# Autodesk Inventor assembly: LIA0002-LID ASSY
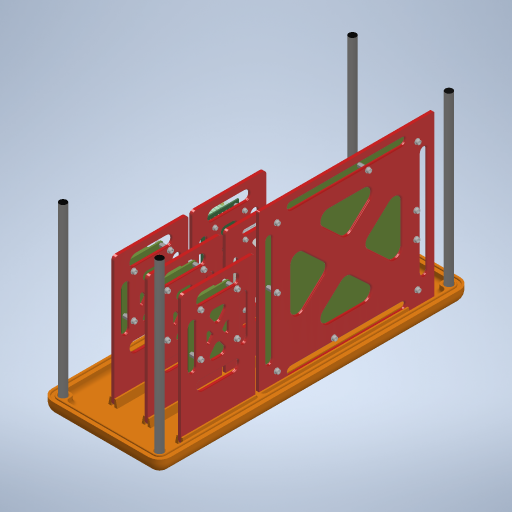
[picture p0: Inventor's stored thumbnail of the model, 512x512]
Saved by Autodesk Inventor 2023 (Build 270158000, 158)
## iProperties
Created: 2023-03-17
Part Number: LIA0002-LID ASSY
Document SubType Name: Assembly
Designer: Louis
Author: Louis
## Documents named in this file (11)
- D:\Louis\Documents\Inventor\Interferometry\LIA0002-LID ASSY.iam
- D:\Louis\Documents\Inventor\Interferometry\LI0002-CASE LID.ipt
- D:\Louis\Documents\Inventor\Interferometry\LIA0001-SHELF.iam
- D:\Louis\Documents\Inventor\Interferometry\LI0004-ROD.ipt
- D:\Louis\Documents\Inventor\Interferometry\LIA0005-IO SHIELD ASSY.iam
- D:\Louis\Documents\Inventor\Interferometry\LI0012-IO SHIELD SEAL.ipt
- D:\Louis\Documents\Inventor\Interferometry\M3 WASHER.ipt
- D:\Louis\Documents\Inventor\Interferometry\M3 X 6.ipt
- D:\Louis\Documents\Inventor\Interferometry\LIA0004-XILINX SHELF ASSY.iam
- D:\Louis\Documents\Inventor\Interferometry\LIA0006-ARDUINO SHELF.iam
- D:\Louis\Documents\Inventor\Interferometry\LIA0007-NETWORKING SHELF.iam
## Components (27 placed, 10 different names)
1. LI0002-CASE LID:1 — Mate:1, Mate:2, Mate:3, Mate:25, Mate:26, Mate:27, Mate:28, Mate:29, Mate:30, Mate:31, Mate:32, Insert:1, Insert:2, Insert:3, Insert:4, Mate:33, Mate:34, Mate:35, Mate:36, Mate:37, Mate:39, Mate:40, Mate:45, Mate:46, Mate:48, Mate:49, Mate:51, Mate:52, Mate:54, Mate:55, Mate:56, Mate:57, Mate:58, Mate:59, Mate:60, Mate:61
2. LI0004-ROD:1 — Mate:26, Mate:30
3. LI0004-ROD:2 — Mate:25, Mate:29
4. LI0004-ROD:3 — Mate:27, Mate:31
5. LI0004-ROD:4 — Mate:28, Mate:32
6. LIA0005-IO SHIELD ASSY:1 [sub-assembly] — Insert:1, Insert:2, Insert:3, Insert:4, Insert:5, Insert:6, Insert:7, Insert:8, Insert:10, Insert:11, Insert:16, Insert:17, Insert:18, Insert:19
7. LI0012-IO SHIELD SEAL:1 — Mate:33, Mate:34, Mate:35
8. M3 WASHER:1 — Insert:6, Insert:12
9. M3 WASHER:3 — Insert:7, Insert:15
10. M3 WASHER:5 — Insert:5, Insert:13
11. M3 WASHER:6 — Insert:8, Insert:14
12. M3 X 6:2 — Insert:10
13. M3 X 6:3 — Insert:12
14. M3 X 6:4 — Insert:11
15. M3 X 6:5 — Insert:13
16. M3 X 6:6 — Insert:14
17. M3 X 6:7 — Insert:15
18. LIA0004-XILINX SHELF ASSY:1 [sub-assembly] — Mate:36, Mate:37, Mate:61
19. LIA0001-SHELF:1 [sub-assembly] — Mate:45, Mate:46, Mate:56
20. LIA0001-SHELF:2 [sub-assembly] — Mate:48, Mate:49, Mate:58
21. LIA0001-SHELF:3 [sub-assembly] — Mate:51, Mate:52, Mate:60
22. LIA0006-ARDUINO SHELF:1 [sub-assembly] — Mate:39, Mate:40, Mate:59
23. M3 X 6:8 — Insert:16
24. M3 X 6:9 — Insert:19
25. M3 X 6:10 — Insert:18
26. M3 X 6:11 — Insert:17
27. LIA0007-NETWORKING SHELF:1 [sub-assembly] — Mate:54, Mate:55, Mate:57
## Relationships (50: Mate 32, Insert 18)
- Mate:1: LI0002-CASE LID:1
- Mate:2: LI0002-CASE LID:1
- Mate:3: LI0002-CASE LID:1
- Mate:25: LI0002-CASE LID:1 ↔ LI0004-ROD:2
- Mate:26: LI0002-CASE LID:1 ↔ LI0004-ROD:1
- Mate:27: LI0002-CASE LID:1 ↔ LI0004-ROD:3
- Mate:28: LI0002-CASE LID:1 ↔ LI0004-ROD:4
- Mate:29: LI0002-CASE LID:1 ↔ LI0004-ROD:2
- Mate:30: LI0002-CASE LID:1 ↔ LI0004-ROD:1
- Mate:31: LI0002-CASE LID:1 ↔ LI0004-ROD:3
- Mate:32: LI0002-CASE LID:1 ↔ LI0004-ROD:4
- Insert:1: LI0002-CASE LID:1 ↔ LIA0005-IO SHIELD ASSY:1
- Insert:2: LI0002-CASE LID:1 ↔ LIA0005-IO SHIELD ASSY:1
- Insert:3: LI0002-CASE LID:1 ↔ LIA0005-IO SHIELD ASSY:1
- Insert:4: LI0002-CASE LID:1 ↔ LIA0005-IO SHIELD ASSY:1
- Mate:33: LI0002-CASE LID:1 ↔ LI0012-IO SHIELD SEAL:1
- Mate:34: LI0002-CASE LID:1 ↔ LI0012-IO SHIELD SEAL:1
- Mate:35: LI0002-CASE LID:1 ↔ LI0012-IO SHIELD SEAL:1
- Insert:5: LIA0005-IO SHIELD ASSY:1 ↔ M3 WASHER:5
- Insert:6: LIA0005-IO SHIELD ASSY:1 ↔ M3 WASHER:1
- Insert:7: LIA0005-IO SHIELD ASSY:1 ↔ M3 WASHER:3
- Insert:8: LIA0005-IO SHIELD ASSY:1 ↔ M3 WASHER:6
- Insert:10: LIA0005-IO SHIELD ASSY:1 ↔ M3 X 6:2
- Insert:11: LIA0005-IO SHIELD ASSY:1 ↔ M3 X 6:4
- Insert:12: M3 WASHER:1 ↔ M3 X 6:3
- Insert:13: M3 WASHER:5 ↔ M3 X 6:5
- Insert:14: M3 WASHER:6 ↔ M3 X 6:6
- Insert:15: M3 WASHER:3 ↔ M3 X 6:7
- Mate:36: LI0002-CASE LID:1 ↔ LIA0004-XILINX SHELF ASSY:1
- Mate:37: LI0002-CASE LID:1 ↔ LIA0004-XILINX SHELF ASSY:1
- Mate:39: LI0002-CASE LID:1 ↔ LIA0006-ARDUINO SHELF:1
- Mate:40: LI0002-CASE LID:1 ↔ LIA0006-ARDUINO SHELF:1
- Mate:45: LI0002-CASE LID:1 ↔ LIA0001-SHELF:1
- Mate:46: LI0002-CASE LID:1 ↔ LIA0001-SHELF:1
- Mate:48: LI0002-CASE LID:1 ↔ LIA0001-SHELF:2
- Mate:49: LI0002-CASE LID:1 ↔ LIA0001-SHELF:2
- Mate:51: LI0002-CASE LID:1 ↔ LIA0001-SHELF:3
- Mate:52: LI0002-CASE LID:1 ↔ LIA0001-SHELF:3
- Insert:16: LIA0005-IO SHIELD ASSY:1 ↔ M3 X 6:8
- Insert:17: LIA0005-IO SHIELD ASSY:1 ↔ M3 X 6:11
- Insert:18: LIA0005-IO SHIELD ASSY:1 ↔ M3 X 6:10
- Insert:19: LIA0005-IO SHIELD ASSY:1 ↔ M3 X 6:9
- Mate:54: LI0002-CASE LID:1 ↔ LIA0007-NETWORKING SHELF:1
- Mate:55: LI0002-CASE LID:1 ↔ LIA0007-NETWORKING SHELF:1
- Mate:56: LI0002-CASE LID:1 ↔ LIA0001-SHELF:1
- Mate:57: LI0002-CASE LID:1 ↔ LIA0007-NETWORKING SHELF:1
- Mate:58: LI0002-CASE LID:1 ↔ LIA0001-SHELF:2
- Mate:59: LI0002-CASE LID:1 ↔ LIA0006-ARDUINO SHELF:1
- Mate:60: LI0002-CASE LID:1 ↔ LIA0001-SHELF:3
- Mate:61: LI0002-CASE LID:1 ↔ LIA0004-XILINX SHELF ASSY:1
